# Autodesk Inventor assembly: Szereles
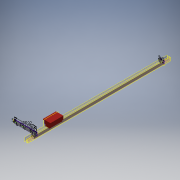
[picture p0: Inventor's stored thumbnail of the model, 180x180]
Saved by Autodesk Inventor 2019 (Build 230136000, 136)
## iProperties
Created: 2022-08-26
Part Number: Szereles
Document SubType Name: Assembly
Designer: laca
Author: laca
## Documents named in this file (4)
- C:\Users\laca\Documents\Inventor\AblakSzuport\Szereles.iam
- C:\Users\laca\Documents\Inventor\AblakSzuport\50x50x5.ipt
- C:\Users\laca\Documents\Inventor\AblakSzuport\AblakProfil.ipt
- C:\Users\laca\Documents\Inventor\AblakSzuport\OldalsoSzuport.ipt
## Components (3 placed, 3 different names)
1. 50x50x5:1 — Mate:1, Flush:1, Mate:2, Flush:5, Flush:6
2. AblakProfil:1 — Mate:1, Flush:1, Flush:2, Flush:3
3. OldalsoSzuport:1 — Flush:3, Mate:2, Flush:4
## Relationships (8: Flush 6, Mate 2)
- Mate:1: 50x50x5:1 ↔ AblakProfil:1
- Flush:1 (-5 mm): 50x50x5:1 ↔ AblakProfil:1
- Flush:2: AblakProfil:1
- Flush:3: AblakProfil:1 ↔ OldalsoSzuport:1
- Mate:2: 50x50x5:1 ↔ OldalsoSzuport:1
- Flush:4: OldalsoSzuport:1
- Flush:5: 50x50x5:1
- Flush:6: 50x50x5:1
